# Autodesk Inventor assembly: 14inLift
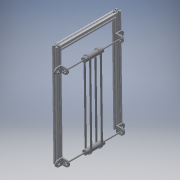
[picture p0: Inventor's stored thumbnail of the model, 180x180]
Saved by Autodesk Inventor 2016 (Build 200138000, 138)
## iProperties
Created: 2016-12-21
Part Number: 14inLift
Document SubType Name: Assembly
Designer: RoboticsUser
Author: RoboticsUser
## Documents named in this file (7)
- C:\Robotics\CAD\2016-17_CAD\14inLift.iam
- C:\Robotics\CAD\2016-17_CAD\LiftLine.ipt
- C:\Robotics\CAD\2016-17_CAD\LiftWireLine14in.ipt
- C:\Robotics\CAD\COTSParts\Bosch Extrusion\Bosch 20x20 16.66 -.ipt
- C:\Robotics\CAD\COTSParts\Actobotics\545 parts\545400_MIR.ipt
- C:\Robotics\CAD\COTSParts\Bosch Extrusion\Bosch 20x20 9 in actual.ipt
- C:\Robotics\CAD\2016-17_CAD\10inax.ipt
## Components (13 placed, 6 different names)
1. LiftLine:1 — Flush:1, Mate:1, Flush:2, Mate:2, Mate:17, Flush:15
2. LiftLine:2 — Mate:3, Flush:3, Mate:15, Mate:16, Flush:14
3. LiftWireLine14in:1 — Flush:1, Mate:1, Mate:3, Flush:3, Flush:11
4. LiftWireLine14in:2 — Flush:2, Mate:2, Mate:15
5. Bosch 20x20 16.66 -:1 — Mate:9, Flush:11, Mate:10, Mate:13, Flush:12, Flush:13
6. Bosch 20x20 16.66 -:2 — Mate:11, Mate:12, Mate:14
7. 545400_MIR:1 — Mate:10, Insert:4
8. 545400_MIR:2 — Mate:9, Insert:2
9. 545400_MIR:3 — Mate:11, Insert:3
10. 545400_MIR:4 — Mate:12, Insert:1
11. Bosch 20x20 9 in actual:1 — Mate:13, Flush:12, Flush:13, Mate:14
12. 10inax:1 — Mate:16, Flush:14, Insert:1, Insert:2
13. 10inax:2 — Mate:17, Flush:15, Insert:3, Insert:4
## Relationships (24: Mate 12, Flush 8, Insert 4)
- Flush:1 (-12.7 mm): LiftLine:1 ↔ LiftWireLine14in:1
- Mate:1: LiftLine:1 ↔ LiftWireLine14in:1
- Flush:2 (-12.7 mm): LiftLine:1 ↔ LiftWireLine14in:2
- Mate:2: LiftLine:1 ↔ LiftWireLine14in:2
- Mate:3: LiftLine:2 ↔ LiftWireLine14in:1
- Flush:3 (-12.7 mm): LiftLine:2 ↔ LiftWireLine14in:1
- Mate:9: Bosch 20x20 16.66 -:1 ↔ 545400_MIR:2
- Flush:11: LiftWireLine14in:1 ↔ Bosch 20x20 16.66 -:1
- Mate:10: Bosch 20x20 16.66 -:1 ↔ 545400_MIR:1
- Mate:11: Bosch 20x20 16.66 -:2 ↔ 545400_MIR:3
- Mate:12: Bosch 20x20 16.66 -:2 ↔ 545400_MIR:4
- Mate:13: Bosch 20x20 16.66 -:1 ↔ Bosch 20x20 9 in actual:1
- Flush:12: Bosch 20x20 16.66 -:1 ↔ Bosch 20x20 9 in actual:1
- Flush:13: Bosch 20x20 16.66 -:1 ↔ Bosch 20x20 9 in actual:1
- Mate:14: Bosch 20x20 16.66 -:2 ↔ Bosch 20x20 9 in actual:1
- Mate:15: LiftLine:2 ↔ LiftWireLine14in:2
- Mate:16: LiftLine:2 ↔ 10inax:1
- Flush:14 (-88.9 mm): LiftLine:2 ↔ 10inax:1
- Insert:1 (-15.24 mm): 545400_MIR:4 ↔ 10inax:1
- Insert:2 (-15.24 mm): 545400_MIR:2 ↔ 10inax:1
- Mate:17: LiftLine:1 ↔ 10inax:2
- Flush:15 (-88.9 mm): LiftLine:1 ↔ 10inax:2
- Insert:3 (-15.24 mm): 545400_MIR:3 ↔ 10inax:2
- Insert:4 (-15.24 mm): 545400_MIR:1 ↔ 10inax:2
